# Autodesk Inventor assembly: arm-asm
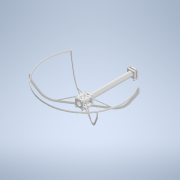
[picture p0: Inventor's stored thumbnail of the model, 180x180]
Saved by Autodesk Inventor 2022 (Build 260153000, 153)
## iProperties
Created: 2020-11-30
Part Number: arm-asm
Document SubType Name: Assembly
Designer: ARRF
Sending System: CREO PARAMETRIC BY PTC INC, 2016510
Preprocessor: CREO PARAMETRIC BY PTC INC, 2016510
Title: JIBI-ASM_ASM
Author: QGLing
Revision Number: 13LAST_VERSION
## Documents named in this file (8)
- C:\Users\ARRF\Desktop\archive_ab8d35b\x500-kit\Frame Models\CAD\Arm\arm-asm.iam
- C:\Users\ARRF\Desktop\archive_ab8d35b\x500-kit\Frame Models\GUAN-JIBI.ipt
- C:\Users\ARRF\Desktop\archive_ab8d35b\x500-kit\Frame Models\JIBI-JIA.ipt
- C:\Users\ARRF\Desktop\archive_ab8d35b\x500-kit\Frame Models\BAN-DJ.ipt
- C:\Users\ARRF\Desktop\archive_ab8d35b\x500-kit\Frame Models\M3-30-PAN-DING.ipt
- C:\Users\ARRF\Desktop\archive_ab8d35b\x500-kit\Frame Models\ZSLM-M3-DING.ipt
- C:\Users\ARRF\Desktop\prop_gurd_l.ipt
- C:\Users\ARRF\Desktop\prop_gurd_r.ipt
## Components (29 placed, 29 different names)
1. 0
2. 1
3. 2
4. 3
5. 4
6. 5
7. 6
8. 7
9. 8
10. 9
11. 10 — Mate:1, Mate:2, Mate:3, Mate:4, Mate:5, Mate:6
12. 11
13. 12
14. 13
15. 14
16. 15
17. 16
18. 17
19. 18
20. 19
21. 20
22. 21
23. 22
24. 23
25. 24
26. 25
27. 26
28. prop_gurd_l:1 — Mate:4, Mate:5, Mate:6
29. prop_gurd_r:1 — Mate:1, Mate:2, Mate:3
## Relationships (6: Mate 6)
- Mate:1: 10 ↔ prop_gurd_r:1
- Mate:2: 10 ↔ prop_gurd_r:1
- Mate:3: 10 ↔ prop_gurd_r:1
- Mate:4: 10 ↔ prop_gurd_l:1
- Mate:5: 10 ↔ prop_gurd_l:1
- Mate:6: 10 ↔ prop_gurd_l:1
